(part 1 of 2)
# Autodesk Inventor assembly: BG001_trajan20_22
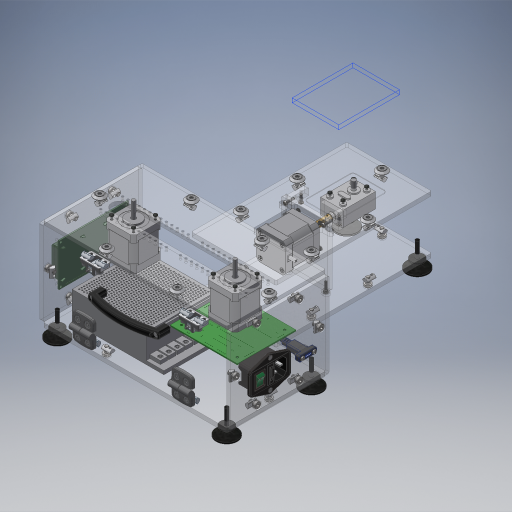
[picture p0: Inventor's stored thumbnail of the model, 512x512]
Saved by Autodesk Inventor 2023 (Build 270158000, 158)
## iProperties
Company: HTBLA Kaindorf
RuleStatus: InUse
Created: 2022-10-30
Part Number: BG001_trajan20_22
Project: Zeichenmaschine_neu
Material: Generisch
Description: Gerüst_mit_Platten
Document SubType Name: Assembly
Designer: trajan20
AfterDocNew0: iProperties-Editor_aufrufen
Author: jan
Keywords: 2022
## Documents named in this file (49)
- C:\Users\eligo\Desktop\DrawMachine\DrawMachineConstruction\inventor\BG001_trajan20_22_Zeichenmaschine_neu_Gerüst_mit_Platten.iam
- C:\Users\eligo\Desktop\DrawMachine\DrawMachineConstruction\inventor\BG000_trajan20_22_Zeichenmaschine_neu_Gestell.iam
- C:\Users\eligo\Desktop\DrawMachine\DrawMachineConstruction\inventor\BT202_trajan20_21_Zeichenmaschine_v2_getriebemotor platte unten.ipt
- C:\Users\eligo\Desktop\DrawMachine\DrawMachineConstruction\inventor\BT201_trajan20_21_Zeichenmaschine_v2_Hauptplatte unten.ipt
- C:\Users\eligo\Desktop\DrawMachine\DrawMachineConstruction\inventor\step Dateien\Steppermotor_NEMA17_17HS19-2004S1_Stepperonline.ipt
- C:\Users\eligo\Desktop\DrawMachine\DrawMachineConstruction\inventor\step Dateien\scharnier_095K2020L00.ipt
- C:\Users\eligo\Desktop\DrawMachine\DrawMachineConstruction\inventor\step Dateien\Magnetschnäpper _093094.ipt
- C:\Users\eligo\Desktop\DrawMachine\DrawMachineConstruction\inventor\step dateien\M4_Nutenstein_096214.ipt
- C:\Users\eligo\Desktop\DrawMachine\DrawMachineConstruction\inventor\BT704_trajan20_21_Zeichenmaschine_v2_Plexi_Zubau_Länge.ipt
- C:\Users\eligo\Desktop\DrawMachine\DrawMachineConstruction\inventor\BT702_trajan20_21_Zeichenmaschine_v2_Plexi_40x80.ipt
- C:\Users\eligo\Desktop\DrawMachine\DrawMachineConstruction\inventor\BT705_trajan20_21_Zeichenmaschine_v2_Plexi_Zubau_Breite.ipt
- C:\Users\eligo\Desktop\DrawMachine\DrawMachineConstruction\inventor\Normteile\de-DE\ISO 14583\ISO 14583 - M2,5x8-4.8.ipt
- C:\Users\eligo\Desktop\DrawMachine\DrawMachineConstruction\inventor\Normteile\de-DE\ISO 14583\ISO 14583 - M2,5x5-4.8.ipt
- C:\Users\eligo\Desktop\DrawMachine\DrawMachineConstruction\inventor\eigene Normteile\Senkschraube DIN 965 M4x8 51305_040_008(High).ipt
- C:\Users\eligo\Desktop\DrawMachine\DrawMachineConstruction\inventor\eigene Normteile\ART 48240 - DIN 6900-1 Z0 T M4x12_0 mm - A2_Steel.ipt
- C:\Users\eligo\Desktop\DrawMachine\DrawMachineConstruction\inventor\step dateien\M5_Nutenstein_096215.ipt
- C:\Users\eligo\Desktop\DrawMachine\DrawMachineConstruction\inventor\Normteile\de-DE\DIN 7984\DIN 7984 - M5 x 8.ipt
- C:\Users\eligo\Desktop\DrawMachine\DrawMachineConstruction\inventor\step dateien\BN 603 1229915 finishing washer M5.ipt
- C:\Users\eligo\Desktop\DrawMachine\DrawMachineConstruction\inventor\eigene Normteile\Senkschraube DIN 965 M5x14 51305_050_014(High).ipt
- C:\Users\eligo\Desktop\DrawMachine\DrawMachineConstruction\inventor\BT706_trajan20_21_Zeichenmaschine_v2_Plexi_Haupt_Display.ipt
- C:\Users\eligo\Desktop\DrawMachine\DrawMachineConstruction\inventor\step Dateien\display_lcd20x4hd44780.ipt
- C:\Users\eligo\Desktop\DrawMachine\DrawMachineConstruction\inventor\BT703_trajan20_21_Zeichenmaschine_v2_Plexi_Tür.ipt
- C:\Users\eligo\Desktop\DrawMachine\DrawMachineConstruction\inventor\BT703_B_trajan20_21_Zeichenmaschine_v2_Griff.ipt
- C:\Users\eligo\Desktop\DrawMachine\DrawMachineConstruction\inventor\Normteile\de-DE\ISO 4762(2)\ISO 4762 - M4 x 16ISO.ipt
- C:\Users\eligo\Desktop\DrawMachine\DrawMachineConstruction\inventor\Normteile\de-DE\AS 1427(03)\AS 1427 - M2 x 4(1).ipt
- C:\Users\eligo\Desktop\DrawMachine\DrawMachineConstruction\inventor\BT003_trajan20_22_Zeichenmaschine_neu_Fuß.ipt
- C:\Users\eligo\Desktop\DrawMachine\DrawMachineConstruction\inventor\BT706_trajan20_21_Zeichenmaschine_v2_Plexi_Haupt_Nothalt.ipt
- C:\Users\eligo\Desktop\DrawMachine\DrawMachineConstruction\inventor\BT801_trajan20_21_Zeichenmaschine_neu_Netzteil.ipt
- C:\Users\eligo\Desktop\DrawMachine\DrawMachineConstruction\inventor\step Dateien\Zeichenmaschine.ipt
- C:\Users\eligo\Desktop\DrawMachine\DrawMachineConstruction\inventor\step Dateien\Type-C Ext CBL - FEMALE +conn.ipt
- C:\Users\eligo\Desktop\DrawMachine\DrawMachineConstruction\inventor\step Dateien\connector-with-switch-and-fuse-3.snapshot.1\baugruppe.iam
- C:\Users\eligo\Desktop\DrawMachine\DrawMachineConstruction\inventor\Normteile\de-DE\AS 1427(03)\AS 1427 - M3 x 5(1).ipt
- C:\Users\eligo\Desktop\DrawMachine\DrawMachineConstruction\inventor\Normteile\de-DE\CNS 9671\CNS 9671 - M3 x 10.ipt
- C:\Users\eligo\Desktop\DrawMachine\DrawMachineConstruction\inventor\von gotzi\BT102_trajan20_21_Zeichenmaschine_v2_Platte Getriebemotor.ipt
- C:\Users\eligo\Desktop\DrawMachine\DrawMachineConstruction\inventor\von gotzi\BT101_trajan20_21_Zeichenmaschine_v2_Platte Stepper Motoren.ipt
- C:\Users\eligo\Desktop\DrawMachine\DrawMachineConstruction\inventor\von gotzi\BT901_goteln20_23_Zeichenmaschine_stepper_getriebe_halterung.ipt
- C:\Users\eligo\Desktop\DrawMachine\DrawMachineConstruction\inventor\Normteile\de-DE\ISO 14583\ISO 14583 - M3x12-4.8.ipt
- C:\Users\eligo\Desktop\DrawMachine\DrawMachineConstruction\inventor\BT902_goteln20_23_Zeichenmaschine_neu_stepper_getriebe_winkel.ipt
- C:\Users\eligo\Desktop\DrawMachine\DrawMachineConstruction\inventor\Normteile\de-DE\ANSI B18.3.4M(2)\ANSI B18.3.4M - M3 x 0.5 x 3(1).ipt
- C:\Users\eligo\Desktop\DrawMachine\DrawMachineConstruction\inventor\Normteile\de-DE\ANSI B18.3.4M(2)\ANSI B18.3.4M - M3 x 0.5 x 10(1).ipt
- C:\Users\eligo\Desktop\DrawMachine\DrawMachineConstruction\inventor\Normteile\de-DE\ANSI B18.3.4M(2)\ANSI B18.3.4M - M3 x 0.5 x 12(1).ipt
- C:\Users\eligo\Desktop\DrawMachine\DrawMachineConstruction\inventor\Normteile\de-DE\ISO 14583\ISO 14583 - M2,5x10-4.8.ipt
- C:\Users\eligo\Desktop\DrawMachine\DrawMachineConstruction\inventor\BT803_goteln20_22_Zeichenmaschine_neu_getriebe.ipt
- C:\Users\eligo\Desktop\DrawMachine\DrawMachineConstruction\inventor\BT804_goteln20_22_Zeichenmaschine_neu_getriebe_lagerung.ipt
- C:\Users\eligo\Desktop\DrawMachine\DrawMachineConstruction\inventor\Normteile\de-DE\DIN BEARING(1)\DIN 625 SKF - SKF 623.ipt
- C:\Users\eligo\Desktop\DrawMachine\DrawMachineConstruction\inventor\BT805_goteln20_22_Zeichenmaschine_neu_getriebe_welle_5zu2.ipt
- C:\Users\eligo\Desktop\DrawMachine\DrawMachineConstruction\inventor\BT805_goteln20_22_Zeichenmaschine_neu_getriebe_welle.ipt
- C:\Users\eligo\Desktop\DrawMachine\DrawMachineConstruction\inventor\Normteile\de-DE\BS 4168(2)\BS 4168 - M2 x 3(2).ipt
- C:\Users\eligo\Desktop\DrawMachine\DrawMachineConstruction\inventor\Normteile\de-DE\BS 4168(2)\BS 4168 - M3 x 2(2).ipt
## Components (172 placed, 48 different names)
1. BT901_goteln20_23_Zeichenmaschine_stepper_getriebe_halterung:1 — Passend:258, Passend:259, Passend:262, Passend:263, Einfügen:44, Einfügen:45, Einfügen:46, Passend:272, Passend:275, Passend:280, Passend:281, Passend:282, Passend:285, Passend:286, Passend:287, Passend:288, Passend:289, Passend:292, Passend:293
2. Schraube ISO 14583:2011(E) M3x12-4.8:1 — Passend:261, Passend:262
3. Schraube ISO 14583:2011(E) M3x12-4.8:2 — Passend:260, Passend:263, Passend:265
4. BT902_goteln20_23_Zeichenmaschine_neu_stepper_getriebe_winkel:1 — Passend:270, Passend:272, Passend:310
5. BT902_goteln20_23_Zeichenmaschine_neu_stepper_getriebe_winkel:2 — Passend:273, Passend:275, Passend:311
6. Linsenschraube mit geschmiedetem Innensechskant - Metrisch M3 x 0.5 x 12:1 — Einfügen:44
7. Linsenschraube mit geschmiedetem Innensechskant - Metrisch M3 x 0.5 x 12:2 — Einfügen:45, Passend:311
8. Linsenschraube mit geschmiedetem Innensechskant - Metrisch M3 x 0.5 x 3:3 — Einfügen:46
9. Linsenschraube mit geschmiedetem Innensechskant - Metrisch M3 x 0.5 x 10:1 — Passend:278, Passend:310
10. Linsenschraube mit geschmiedetem Innensechskant - Metrisch M3 x 0.5 x 10:2 — Passend:277
11. Steppermotor_NEMA17_17HS19-2004S1_Stepperonline:3 — Passend:280, Passend:283, Passend:284, Passend:290, Passend:291, Passend:300, Passend:304, Passend:305
12. Schraube ISO 14583:2011(E) M2,5x10-4.8:1 — Passend:281, Passend:282, Passend:283
13. Schraube ISO 14583:2011(E) M2,5x10-4.8:2 — Passend:288, Passend:291, Passend:293
14. Schraube ISO 14583:2011(E) M2,5x10-4.8:3 — Passend:284, Passend:285, Passend:286, Passend:287
15. Schraube ISO 14583:2011(E) M2,5x10-4.8:4 — Passend:289, Passend:290, Passend:292
16. BT803_goteln20_22_Zeichenmaschine_neu_getriebe:1 — Passend:294, Passend:295, Passend:296, Passend:297, Passend:298, Passend:300, Fluchtend:16, Fluchtend:17, Passend:301
17. BT804_goteln20_22_Zeichenmaschine_neu_getriebe_lagerung:1 — Fluchtend:16, Fluchtend:17, Passend:301, Einfügen:47
18. DIN 625 SKF SKF 623:1 — Einfügen:47, Passend:302, Passend:303
19. BT805_goteln20_22_Zeichenmaschine_neu_getriebe_welle_5zu2:1 — Passend:302, Passend:303, Passend:304, Passend:306, Passend:307, Passend:308, Fluchtend:18
20. BS 4168 : Teil 2 Innensechskantschrauben und Stiftschlüssel, metrische Ausführung - Spezifikation für Sechskant-Gewindestifte mit Kegelstumpf - Metrisch M3 x 2:1 — Passend:305, Passend:306
21. BS 4168 : Teil 2 Innensechskantschrauben und Stiftschlüssel, metrische Ausführung - Spezifikation für Sechskant-Gewindestifte mit Kegelstumpf - Metrisch M2 x 3:1 — Passend:307, Passend:309
22. BT805_goteln20_22_Zeichenmaschine_neu_getriebe_welle:1 — Passend:308, Fluchtend:18, Passend:309
23. BT003_trajan20_22_Zeichenmaschine_neu_Fuß:1 — Passend:205, Passend:206
24. BT003_trajan20_22_Zeichenmaschine_neu_Fuß:2 — Passend:209, Passend:211
25. BT003_trajan20_22_Zeichenmaschine_neu_Fuß:3 — Passend:207, Passend:210
26. BT003_trajan20_22_Zeichenmaschine_neu_Fuß:4 — Passend:208, Passend:212
27. BT003_trajan20_22_Zeichenmaschine_neu_Fuß:5 — Passend:214, Passend:216
28. BT003_trajan20_22_Zeichenmaschine_neu_Fuß:6 — Passend:213, Passend:215
29. BG000_trajan20_22_Zeichenmaschine_neu_Gestell:1 [sub-assembly] — Passend:2, Fluchtend:3, Fluchtend:4, Passend:3, Fluchtend:5, Fluchtend:6, Passend:14, Passend:15, Passend:16, Passend:17, Passend:18, Passend:19, Passend:20, Winkel:1, Passend:21, Passend:22, Passend:23, Passend:24, Passend:25, Passend:26, Passend:27, Passend:28, Passend:29, Passend:30, Passend:31, Passend:32, Passend:33, Passend:34, Passend:35, Passend:36, Passend:37, Passend:38, Passend:39, Passend:40, Passend:41, Passend:43, Winkel:2, Passend:45, Passend:46, Winkel:3, Winkel:4, Passend:49, Passend:50, Passend:51, Passend:52, Winkel:5, Winkel:6, Winkel:7, Winkel:8, Fluchtend:10, Fluchtend:11, Passend:74, Passend:75, Passend:76, Passend:77, Passend:85, Winkel:9, Passend:86, Passend:87, Winkel:10, Winkel:11, Passend:88, Passend:89, Winkel:12, Winkel:13, Passend:90, Winkel:14, Passend:97, Passend:98, Passend:99, Passend:100, Passend:101, Winkel:15, Winkel:16, Winkel:17, Winkel:18, Winkel:19, Passend:107, Winkel:20, Passend:108, Passend:109, Passend:110, Passend:111, Passend:112, Winkel:21, Winkel:22, Winkel:23, Winkel:24, Winkel:25, Passend:119, Winkel:26, Passend:120, Passend:121, Passend:122, Passend:123, Winkel:27, Winkel:28, Winkel:29, Winkel:30, Passend:173, Fluchtend:12, Fluchtend:13, Winkel:31, Passend:176, Passend:177, Passend:178, Passend:179, Passend:180, Passend:181, Winkel:32, Winkel:33, Winkel:34, Winkel:35, Winkel:36, Winkel:37, Passend:206, Passend:210, Passend:211, Passend:212, Passend:215, Passend:216, Passend:217, Fluchtend:14, Fluchtend:15, Passend:219, Passend:220, Passend:221, Passend:222, Passend:223, Passend:224, Passend:225, Passend:226, Winkel:38, Winkel:39, Winkel:40, Winkel:41, Winkel:42, Winkel:43, Passend:235, Passend:245
30. BT704_trajan20_21_Zeichenmaschine_v2_Plexi_Zubau_Länge:1 — Passend:27, Passend:28, Passend:29
31. BT702_trajan20_21_Zeichenmaschine_v2_Plexi_40x80:1 — Passend:33, Passend:34, Passend:35
32. BT702_trajan20_21_Zeichenmaschine_v2_Plexi_40x80:2 — Passend:36, Passend:37, Passend:38
33. BT705_trajan20_21_Zeichenmaschine_v2_Plexi_Zubau_Breite:1 — Passend:39, Passend:40, Passend:41
34. BT704_trajan20_21_Zeichenmaschine_v2_Plexi_Zubau_Länge:2 — Passend:30, Passend:31, Passend:32
35. Steppermotor_NEMA17_17HS19-2004S1_Stepperonline:2 — Passend:254, Passend:255
36. Steppermotor_NEMA17_17HS19-2004S1_Stepperonline:1 — Passend:256, Passend:257
37. Schraube ISO 14583:2011(E) M2,5x8-4.8:1 — Einfügen:36, Passend:257
38. Schraube ISO 14583:2011(E) M2,5x8-4.8:2 — Einfügen:37
39. Schraube ISO 14583:2011(E) M2,5x8-4.8:3 — Einfügen:38, Passend:256
40. Schraube ISO 14583:2011(E) M2,5x8-4.8:4 — Einfügen:39
41. Schraube ISO 14583:2011(E) M2,5x8-4.8:5 — Einfügen:40, Passend:254
42. Schraube ISO 14583:2011(E) M2,5x8-4.8:8 — Einfügen:41
43. Schraube ISO 14583:2011(E) M2,5x8-4.8:7 — Einfügen:42, Passend:255
44. Schraube ISO 14583:2011(E) M2,5x8-4.8:6 — Einfügen:43
45. Schraube ISO 14583:2011(E) M2,5x5-4.8:1 — Passend:249, Passend:253, Passend:296
46. Schraube ISO 14583:2011(E) M2,5x5-4.8:2 — Passend:252, Passend:295
47. Schraube ISO 14583:2011(E) M2,5x5-4.8:3 — Passend:251, Passend:299
48. Schraube ISO 14583:2011(E) M2,5x5-4.8:4 — Passend:250, Passend:298
49. Senkschraube DIN 965 M4x8 51305_040_008(High):1 — Passend:65, Passend:72
50. Senkschraube DIN 965 M4x8 51305_040_008(High):2 — Passend:66, Passend:71
51. Senkschraube DIN 965 M4x8 51305_040_008(High):3 — Passend:67, Passend:70
52. Senkschraube DIN 965 M4x8 51305_040_008(High):4 — Passend:68, Passend:69
53. scharnier_095K2020L00:2 — Passend:15, Passend:23, Passend:24, Passend:25, Passend:47, Passend:48, Passend:65, Passend:66, Passend:71, Passend:72, Passend:188, Passend:191, Passend:196, Passend:197
54. scharnier_095K2020L00:1 — Passend:14, Passend:21, Passend:22, Passend:26, Passend:42, Passend:44, Passend:67, Passend:68, Passend:69, Passend:70, Passend:190, Passend:198, Passend:199
55. M4_Nutenstein_096214:4 — Passend:46, Winkel:3, Passend:48
56. M4_Nutenstein_096214:3 — Passend:45, Winkel:4, Passend:47
57. M4_Nutenstein_096214:2 — Passend:43, Winkel:2, Passend:44
58. M4_Nutenstein_096214:1 — Passend:20, Winkel:1, Passend:42
59. M4_Nutenstein_096214:8 — Passend:52, Winkel:5, Passend:56, Passend:77, Passend:83
60. M4_Nutenstein_096214:5 — Passend:49, Winkel:7, Passend:53, Passend:73, Passend:74
61. M4_Nutenstein_096214:6 — Passend:50, Winkel:8, Passend:54, Passend:75, Passend:78
62. M4_Nutenstein_096214:7 — Passend:51, Winkel:6, Passend:55, Passend:76, Passend:81
63. Magnetschnäpper _093094:2 — Passend:16, Passend:18, Passend:55, Passend:56, Fluchtend:11, Passend:82, Passend:84
64. Magnetschnäpper _093094:1 — Passend:17, Passend:19, Passend:53, Passend:54, Fluchtend:10, Passend:79, Passend:80
65. ART 48240 - DIN 6900-1 Z0 T M4x12_0 mm - A2_Steel:1 — Passend:73, Passend:80
66. ART 48240 - DIN 6900-1 Z0 T M4x12_0 mm - A2_Steel:2 — Passend:78, Passend:79
67. ART 48240 - DIN 6900-1 Z0 T M4x12_0 mm - A2_Steel:3 — Passend:81, Passend:82
68. ART 48240 - DIN 6900-1 Z0 T M4x12_0 mm - A2_Steel:4 — Passend:83, Passend:84
69. BT101_trajan20_21_Zeichenmaschine_v2_Platte Stepper Motoren:2 — Einfügen:36, Einfügen:37, Einfügen:38, Einfügen:39, Einfügen:40, Einfügen:41, Einfügen:42, Einfügen:43
70. M5_Nutenstein_096215:1 — Passend:85, Winkel:9
71. M5_Nutenstein_096215:2 — Passend:86, Winkel:11
72. M5_Nutenstein_096215:3 — Passend:87, Winkel:10
73. M5_Nutenstein_096215:4 — Passend:89, Winkel:12
74. M5_Nutenstein_096215:5 — Passend:88, Winkel:13
75. M5_Nutenstein_096215:6 — Passend:90, Winkel:14
76. BN 603 1229915 finishing washer M5:1 — Passend:147
77. BN 603 1229915 finishing washer M5:2 — Passend:148
78. BN 603 1229915 finishing washer M5:3 — Passend:150
79. BN 603 1229915 finishing washer M5:4 — Passend:149
80. BN 603 1229915 finishing washer M5:5 — Passend:151
81. BN 603 1229915 finishing washer M5:6 — Passend:152
82. Senkschraube DIN 965 M5x14 51305_050_014(High):1 — Passend:148
83. Senkschraube DIN 965 M5x14 51305_050_014(High):2 — Passend:149
84. Senkschraube DIN 965 M5x14 51305_050_014(High):3 — Passend:150
85. Senkschraube DIN 965 M5x14 51305_050_014(High):4 — Passend:151
86. Senkschraube DIN 965 M5x14 51305_050_014(High):5 — Passend:152
87. Senkschraube DIN 965 M5x14 51305_050_014(High):6 — Passend:147
88. BT102_trajan20_21_Zeichenmaschine_v2_Platte Getriebemotor:2 — Passend:246, Passend:247, Passend:248, Passend:249, Passend:250, Passend:251, Passend:252, Passend:253, Passend:259, Passend:270, Passend:273, Passend:277, Passend:278, Passend:294, Passend:297, Passend:299
89. M5_Nutenstein_096215:7 — Passend:97, Winkel:17, Passend:246, Passend:247
90. M5_Nutenstein_096215:8 — Passend:98, Winkel:18
91. M5_Nutenstein_096215:9 — Passend:99, Winkel:19
92. M5_Nutenstein_096215:10 — Passend:100, Winkel:16
93. M5_Nutenstein_096215:11 — Passend:101, Winkel:15
94. BN 603 1229915 finishing washer M5:7 — Passend:169
95. BN 603 1229915 finishing washer M5:8 — Passend:172
96. BN 603 1229915 finishing washer M5:9 — Passend:171
97. BN 603 1229915 finishing washer M5:10 — Passend:170
98. BN 603 1229915 finishing washer M5:11 — Passend:168
99. Senkschraube DIN 965 M5x14 51305_050_014(High):7 — Passend:172
100. Senkschraube DIN 965 M5x14 51305_050_014(High):8 — Passend:171
101. Senkschraube DIN 965 M5x14 51305_050_014(High):9 — Passend:170, Passend:248
102. Senkschraube DIN 965 M5x14 51305_050_014(High):10 — Passend:169
103. Senkschraube DIN 965 M5x14 51305_050_014(High):11 — Passend:168
104. BT201_trajan20_21_Zeichenmaschine_v2_Hauptplatte unten:1 — Passend:3, Fluchtend:5, Fluchtend:6, Passend:113, Passend:114, Passend:115, Passend:116, Passend:117, Passend:118, Einfügen:9, Einfügen:10, Einfügen:11, Einfügen:12, Einfügen:13, Einfügen:14, Passend:205, Passend:207, Passend:208, Passend:209, Passend:218, Passend:233
105. M5_Nutenstein_096215:12 — Passend:107, Winkel:20, Passend:114
106. M5_Nutenstein_096215:13 — Passend:108, Winkel:24, Passend:118
107. M5_Nutenstein_096215:14 — Passend:109, Winkel:23, Passend:117
108. M5_Nutenstein_096215:15 — Passend:110, Winkel:25, Passend:113
109. M5_Nutenstein_096215:16 — Passend:111, Winkel:21, Passend:116
110. M5_Nutenstein_096215:17 — Passend:112, Winkel:22, Passend:115
111. DIN 7984 M5 x 8:1 — Einfügen:9
112. DIN 7984 M5 x 8:2 — Einfügen:10
113. DIN 7984 M5 x 8:3 — Einfügen:11
114. DIN 7984 M5 x 8:4 — Einfügen:12
115. DIN 7984 M5 x 8:5 — Einfügen:13
116. DIN 7984 M5 x 8:6 — Einfügen:14
117. BT202_trajan20_21_Zeichenmaschine_v2_getriebemotor platte unten:1 — Passend:2, Fluchtend:3, Fluchtend:4, Passend:124, Passend:125, Passend:126, Passend:127, Passend:128, Einfügen:15, Einfügen:16, Einfügen:17, Einfügen:18, Einfügen:19, Passend:213, Passend:214, Passend:258, Passend:260, Passend:261, Passend:264, Winkel:44
118. M5_Nutenstein_096215:18 — Passend:119, Winkel:26, Passend:124
119. M5_Nutenstein_096215:19 — Passend:120, Winkel:29, Passend:126
120. M5_Nutenstein_096215:20 — Passend:121, Winkel:30, Passend:128
121. M5_Nutenstein_096215:21 — Passend:123, Winkel:28, Passend:127
122. M5_Nutenstein_096215:22 — Passend:122, Winkel:27, Passend:125
123. DIN 7984 M5 x 8:7 — Einfügen:15
124. DIN 7984 M5 x 8:8 — Einfügen:16
125. DIN 7984 M5 x 8:9 — Einfügen:17
126. DIN 7984 M5 x 8:10 — Einfügen:18
127. DIN 7984 M5 x 8:11 — Einfügen:19
128. BT706_trajan20_21_Zeichenmaschine_v2_Plexi_Haupt_Display:1 — Passend:173, Fluchtend:12, Fluchtend:13, Passend:174, Passend:175, Passend:182, Passend:183, Passend:184, Passend:185, Passend:186, Passend:187, Einfügen:20, Einfügen:21, Einfügen:22, Einfügen:23, Einfügen:24, Einfügen:25
129. display_lcd20x4hd44780:1 — Passend:174, Passend:175, Winkel:31
130. M5_Nutenstein_096215:23 — Passend:176, Winkel:37, Passend:182
131. M5_Nutenstein_096215:24 — Passend:177, Winkel:35, Passend:187
132. M5_Nutenstein_096215:25 — Passend:178, Winkel:34, Passend:186
133. M5_Nutenstein_096215:26 — Passend:179, Winkel:36, Passend:185
134. M5_Nutenstein_096215:27 — Passend:181, Winkel:32, Passend:183
135. M5_Nutenstein_096215:28 — Passend:180, Winkel:33, Passend:184
136. DIN 7984 M5 x 8:12 — Einfügen:20
137. DIN 7984 M5 x 8:13 — Einfügen:21
138. DIN 7984 M5 x 8:14 — Einfügen:22
139. DIN 7984 M5 x 8:15 — Einfügen:23
140. DIN 7984 M5 x 8:16 — Einfügen:24
141. DIN 7984 M5 x 8:17 — Einfügen:25
142. BT703_trajan20_21_Zeichenmaschine_v2_Plexi_Tür:1 — Passend:188, Passend:190, Passend:191, Passend:192, Passend:193, Passend:194, Passend:195, Passend:200, Passend:201, Passend:202, Passend:203, Passend:204
143. BT703_B_trajan20_21_Zeichenmaschine_v2_Griff:1 — Passend:200, Passend:201, Passend:202, Einfügen:26, Einfügen:27
144. Senkschraube DIN 965 M4x8 51305_040_008(High):5 — Passend:192, Passend:198
145. Senkschraube DIN 965 M4x8 51305_040_008(High):6 — Passend:193, Passend:199
146. Senkschraube DIN 965 M4x8 51305_040_008(High):7 — Passend:194, Passend:196
147. Senkschraube DIN 965 M4x8 51305_040_008(High):8 — Passend:195, Passend:197
148. ISO 4762 M4 x 16:1 — Einfügen:26
149. ISO 4762 M4 x 16:2 — Einfügen:27
150. AS 1427 - Metrisch M2 x 4:1 — Passend:203
151. AS 1427 - Metrisch M2 x 4:2 — Passend:204
152. BT706_trajan20_21_Zeichenmaschine_v2_Plexi_Haupt_Nothalt:1 — Passend:217, Fluchtend:14, Fluchtend:15, Passend:227, Passend:228, Passend:229, Passend:230, Passend:231, Passend:232, Einfügen:28, Einfügen:29, Einfügen:30, Einfügen:31, Einfügen:32, Einfügen:33, Passend:236, Passend:237, Passend:239, Passend:240, Passend:241, Passend:244
153. M5_Nutenstein_096215:29 — Passend:221, Winkel:42, Passend:227
154. M5_Nutenstein_096215:30 — Passend:224, Winkel:40, Passend:231
155. M5_Nutenstein_096215:31 — Passend:225, Winkel:41, Passend:232
156. M5_Nutenstein_096215:32 — Passend:223, Winkel:39, Passend:229
157. M5_Nutenstein_096215:33 — Passend:222, Winkel:38, Passend:228
158. M5_Nutenstein_096215:34 — Passend:226, Winkel:43, Passend:230
159. DIN 7984 M5 x 8:23 — Einfügen:33
160. DIN 7984 M5 x 8:18 — Einfügen:28
161. DIN 7984 M5 x 8:19 — Einfügen:29
162. DIN 7984 M5 x 8:20 — Einfügen:30
163. DIN 7984 M5 x 8:21 — Einfügen:31
164. DIN 7984 M5 x 8:22 — Einfügen:32
165. Type-C Ext CBL - FEMALE +conn:1 — Passend:239, Passend:240, Passend:241, Einfügen:34, Einfügen:35
166. baugruppe:1 [sub-assembly] — Passend:236, Passend:237, Passend:242, Passend:243, Passend:244
167. AS 1427 - Metrisch M3 x 5:1 — Passend:242
168. AS 1427 - Metrisch M3 x 5:2 — Passend:243
169. CNS 9671 M3 x 10:1 — Einfügen:34
170. CNS 9671 M3 x 10:2 — Einfügen:35
171. Zeichenmaschine:1 — Passend:233, Passend:235, Passend:245
172. BT801_trajan20_21_Zeichenmaschine_neu_Netzteil:1 — Passend:218, Passend:219, Passend:220
## Relationships (382: Mate 282, Angle 44, Insert 39, Flush 17)
- [Mate]: BG000_trajan20_22_Zeichenmaschine_neu_Gestell:1 ↔ BT101_trajan20_21_Zeichenmaschine_v2_Platte Stepper Motoren:2
- [Flush]: BG000_trajan20_22_Zeichenmaschine_neu_Gestell:1 ↔ BT101_trajan20_21_Zeichenmaschine_v2_Platte Stepper Motoren:2
- [Flush]: BG000_trajan20_22_Zeichenmaschine_neu_Gestell:1 ↔ BT101_trajan20_21_Zeichenmaschine_v2_Platte Stepper Motoren:2
- Passend:2 [Mate]: BG000_trajan20_22_Zeichenmaschine_neu_Gestell:1 ↔ BT202_trajan20_21_Zeichenmaschine_v2_getriebemotor platte unten:1
- Fluchtend:3 [Flush]: BG000_trajan20_22_Zeichenmaschine_neu_Gestell:1 ↔ BT202_trajan20_21_Zeichenmaschine_v2_getriebemotor platte unten:1
- Fluchtend:4 [Flush]: BG000_trajan20_22_Zeichenmaschine_neu_Gestell:1 ↔ BT202_trajan20_21_Zeichenmaschine_v2_getriebemotor platte unten:1
- Passend:3 [Mate]: BG000_trajan20_22_Zeichenmaschine_neu_Gestell:1 ↔ BT201_trajan20_21_Zeichenmaschine_v2_Hauptplatte unten:1
- Fluchtend:5 [Flush]: BG000_trajan20_22_Zeichenmaschine_neu_Gestell:1 ↔ BT201_trajan20_21_Zeichenmaschine_v2_Hauptplatte unten:1
- Fluchtend:6 [Flush]: BG000_trajan20_22_Zeichenmaschine_neu_Gestell:1 ↔ BT201_trajan20_21_Zeichenmaschine_v2_Hauptplatte unten:1
- [Mate]: BG000_trajan20_22_Zeichenmaschine_neu_Gestell:1 ↔ BT102_trajan20_21_Zeichenmaschine_v2_Platte Getriebemotor:2
- [Flush]: BG000_trajan20_22_Zeichenmaschine_neu_Gestell:1 ↔ BT102_trajan20_21_Zeichenmaschine_v2_Platte Getriebemotor:2
- [Flush]: BG000_trajan20_22_Zeichenmaschine_neu_Gestell:1 ↔ BT102_trajan20_21_Zeichenmaschine_v2_Platte Getriebemotor:2
- [Mate]: Steppermotor_NEMA17_17HS19-2004S1_Stepperonline:2 ↔ BT101_trajan20_21_Zeichenmaschine_v2_Platte Stepper Motoren:2
- [Mate]: Steppermotor_NEMA17_17HS19-2004S1_Stepperonline:1 ↔ BT101_trajan20_21_Zeichenmaschine_v2_Platte Stepper Motoren:2
- Passend:14 [Mate]: BG000_trajan20_22_Zeichenmaschine_neu_Gestell:1 ↔ scharnier_095K2020L00:1
- Passend:15 [Mate]: BG000_trajan20_22_Zeichenmaschine_neu_Gestell:1 ↔ scharnier_095K2020L00:2
- Passend:16 [Mate]: BG000_trajan20_22_Zeichenmaschine_neu_Gestell:1 ↔ Magnetschnäpper _093094:2
- Passend:17 [Mate]: BG000_trajan20_22_Zeichenmaschine_neu_Gestell:1 ↔ Magnetschnäpper _093094:1
- Passend:18 [Mate] (26 mm): BG000_trajan20_22_Zeichenmaschine_neu_Gestell:1 ↔ Magnetschnäpper _093094:2
- Passend:19 [Mate] (26 mm): BG000_trajan20_22_Zeichenmaschine_neu_Gestell:1 ↔ Magnetschnäpper _093094:1
- Passend:20 [Mate] (0.55 mm): BG000_trajan20_22_Zeichenmaschine_neu_Gestell:1 ↔ M4_Nutenstein_096214:1
- Winkel:1 [Angle] (0 deg): BG000_trajan20_22_Zeichenmaschine_neu_Gestell:1 ↔ M4_Nutenstein_096214:1
- Passend:21 [Mate] (2.5 mm): BG000_trajan20_22_Zeichenmaschine_neu_Gestell:1 ↔ scharnier_095K2020L00:1
- Passend:22 [Mate] (2.5 mm): BG000_trajan20_22_Zeichenmaschine_neu_Gestell:1 ↔ scharnier_095K2020L00:1
- Passend:23 [Mate] (2.5 mm): BG000_trajan20_22_Zeichenmaschine_neu_Gestell:1 ↔ scharnier_095K2020L00:2
- Passend:24 [Mate] (2.5 mm): BG000_trajan20_22_Zeichenmaschine_neu_Gestell:1 ↔ scharnier_095K2020L00:2
- Passend:25 [Mate] (40 mm): BG000_trajan20_22_Zeichenmaschine_neu_Gestell:1 ↔ scharnier_095K2020L00:2
- Passend:26 [Mate] (40 mm): BG000_trajan20_22_Zeichenmaschine_neu_Gestell:1 ↔ scharnier_095K2020L00:1
- Passend:27 [Mate]: BG000_trajan20_22_Zeichenmaschine_neu_Gestell:1 ↔ BT704_trajan20_21_Zeichenmaschine_v2_Plexi_Zubau_Länge:1
- Passend:28 [Mate] (0.5 mm): BG000_trajan20_22_Zeichenmaschine_neu_Gestell:1 ↔ BT704_trajan20_21_Zeichenmaschine_v2_Plexi_Zubau_Länge:1
- Passend:29 [Mate] (0.5 mm): BG000_trajan20_22_Zeichenmaschine_neu_Gestell:1 ↔ BT704_trajan20_21_Zeichenmaschine_v2_Plexi_Zubau_Länge:1
- Passend:30 [Mate]: BG000_trajan20_22_Zeichenmaschine_neu_Gestell:1 ↔ BT704_trajan20_21_Zeichenmaschine_v2_Plexi_Zubau_Länge:2
- Passend:31 [Mate] (0.5 mm): BG000_trajan20_22_Zeichenmaschine_neu_Gestell:1 ↔ BT704_trajan20_21_Zeichenmaschine_v2_Plexi_Zubau_Länge:2
- Passend:32 [Mate] (0.5 mm): BG000_trajan20_22_Zeichenmaschine_neu_Gestell:1 ↔ BT704_trajan20_21_Zeichenmaschine_v2_Plexi_Zubau_Länge:2
- Passend:33 [Mate]: BG000_trajan20_22_Zeichenmaschine_neu_Gestell:1 ↔ BT702_trajan20_21_Zeichenmaschine_v2_Plexi_40x80:1
- Passend:34 [Mate] (0.5 mm): BG000_trajan20_22_Zeichenmaschine_neu_Gestell:1 ↔ BT702_trajan20_21_Zeichenmaschine_v2_Plexi_40x80:1
- Passend:35 [Mate] (0.5 mm): BG000_trajan20_22_Zeichenmaschine_neu_Gestell:1 ↔ BT702_trajan20_21_Zeichenmaschine_v2_Plexi_40x80:1
- Passend:36 [Mate]: BG000_trajan20_22_Zeichenmaschine_neu_Gestell:1 ↔ BT702_trajan20_21_Zeichenmaschine_v2_Plexi_40x80:2
- Passend:37 [Mate] (0.5 mm): BG000_trajan20_22_Zeichenmaschine_neu_Gestell:1 ↔ BT702_trajan20_21_Zeichenmaschine_v2_Plexi_40x80:2
- Passend:38 [Mate] (0.5 mm): BG000_trajan20_22_Zeichenmaschine_neu_Gestell:1 ↔ BT702_trajan20_21_Zeichenmaschine_v2_Plexi_40x80:2
- Passend:39 [Mate]: BG000_trajan20_22_Zeichenmaschine_neu_Gestell:1 ↔ BT705_trajan20_21_Zeichenmaschine_v2_Plexi_Zubau_Breite:1
- Passend:40 [Mate] (0.5 mm): BG000_trajan20_22_Zeichenmaschine_neu_Gestell:1 ↔ BT705_trajan20_21_Zeichenmaschine_v2_Plexi_Zubau_Breite:1
- Passend:41 [Mate] (0.5 mm): BG000_trajan20_22_Zeichenmaschine_neu_Gestell:1 ↔ BT705_trajan20_21_Zeichenmaschine_v2_Plexi_Zubau_Breite:1
- Passend:42 [Mate]: scharnier_095K2020L00:1 ↔ M4_Nutenstein_096214:1
- Passend:43 [Mate] (0.55 mm): BG000_trajan20_22_Zeichenmaschine_neu_Gestell:1 ↔ M4_Nutenstein_096214:2
- Winkel:2 [Angle] (0 deg): BG000_trajan20_22_Zeichenmaschine_neu_Gestell:1 ↔ M4_Nutenstein_096214:2
- Passend:44 [Mate]: scharnier_095K2020L00:1 ↔ M4_Nutenstein_096214:2
- Passend:45 [Mate] (0.55 mm): BG000_trajan20_22_Zeichenmaschine_neu_Gestell:1 ↔ M4_Nutenstein_096214:3
- Passend:46 [Mate] (0.55 mm): BG000_trajan20_22_Zeichenmaschine_neu_Gestell:1 ↔ M4_Nutenstein_096214:4
- Winkel:3 [Angle] (0 deg): BG000_trajan20_22_Zeichenmaschine_neu_Gestell:1 ↔ M4_Nutenstein_096214:4
- Winkel:4 [Angle] (0 deg): BG000_trajan20_22_Zeichenmaschine_neu_Gestell:1 ↔ M4_Nutenstein_096214:3
- Passend:47 [Mate]: scharnier_095K2020L00:2 ↔ M4_Nutenstein_096214:3
- Passend:48 [Mate]: scharnier_095K2020L00:2 ↔ M4_Nutenstein_096214:4
- Passend:49 [Mate] (0.55 mm): BG000_trajan20_22_Zeichenmaschine_neu_Gestell:1 ↔ M4_Nutenstein_096214:5
- Passend:50 [Mate] (0.55 mm): BG000_trajan20_22_Zeichenmaschine_neu_Gestell:1 ↔ M4_Nutenstein_096214:6
- Passend:51 [Mate] (0.55 mm): BG000_trajan20_22_Zeichenmaschine_neu_Gestell:1 ↔ M4_Nutenstein_096214:7
- Passend:52 [Mate] (0.55 mm): BG000_trajan20_22_Zeichenmaschine_neu_Gestell:1 ↔ M4_Nutenstein_096214:8
- Winkel:5 [Angle] (0 deg): BG000_trajan20_22_Zeichenmaschine_neu_Gestell:1 ↔ M4_Nutenstein_096214:8
- Winkel:6 [Angle] (0 deg): BG000_trajan20_22_Zeichenmaschine_neu_Gestell:1 ↔ M4_Nutenstein_096214:7
- Winkel:7 [Angle] (0 deg): BG000_trajan20_22_Zeichenmaschine_neu_Gestell:1 ↔ M4_Nutenstein_096214:5
- Winkel:8 [Angle] (0 deg): BG000_trajan20_22_Zeichenmaschine_neu_Gestell:1 ↔ M4_Nutenstein_096214:6
- Passend:53 [Mate] (2.15 mm): M4_Nutenstein_096214:5 ↔ Magnetschnäpper _093094:1
- Passend:54 [Mate] (2.15 mm): M4_Nutenstein_096214:6 ↔ Magnetschnäpper _093094:1
- Passend:55 [Mate] (2.15 mm): M4_Nutenstein_096214:7 ↔ Magnetschnäpper _093094:2
- Passend:56 [Mate] (2.15 mm): M4_Nutenstein_096214:8 ↔ Magnetschnäpper _093094:2
- Passend:65 [Mate]: Senkschraube DIN 965 M4x8 51305_040_008(High):1 ↔ scharnier_095K2020L00:2
- Passend:66 [Mate]: Senkschraube DIN 965 M4x8 51305_040_008(High):2 ↔ scharnier_095K2020L00:2
- Passend:67 [Mate]: Senkschraube DIN 965 M4x8 51305_040_008(High):3 ↔ scharnier_095K2020L00:1
- Passend:68 [Mate]: Senkschraube DIN 965 M4x8 51305_040_008(High):4 ↔ scharnier_095K2020L00:1
- Passend:69 [Mate]: Senkschraube DIN 965 M4x8 51305_040_008(High):4 ↔ scharnier_095K2020L00:1
- Passend:70 [Mate]: Senkschraube DIN 965 M4x8 51305_040_008(High):3 ↔ scharnier_095K2020L00:1
- Passend:71 [Mate]: Senkschraube DIN 965 M4x8 51305_040_008(High):2 ↔ scharnier_095K2020L00:2
- Passend:72 [Mate]: Senkschraube DIN 965 M4x8 51305_040_008(High):1 ↔ scharnier_095K2020L00:2
- Passend:73 [Mate]: M4_Nutenstein_096214:5 ↔ ART 48240 - DIN 6900-1 Z0 T M4x12_0 mm - A2_Steel:1
- Fluchtend:10 [Flush] (5 mm): BG000_trajan20_22_Zeichenmaschine_neu_Gestell:1 ↔ Magnetschnäpper _093094:1
- Fluchtend:11 [Flush] (5 mm): BG000_trajan20_22_Zeichenmaschine_neu_Gestell:1 ↔ Magnetschnäpper _093094:2
- Passend:74 [Mate] (2.5 mm): BG000_trajan20_22_Zeichenmaschine_neu_Gestell:1 ↔ M4_Nutenstein_096214:5
- Passend:75 [Mate] (2.5 mm): BG000_trajan20_22_Zeichenmaschine_neu_Gestell:1 ↔ M4_Nutenstein_096214:6
- Passend:76 [Mate] (2.5 mm): BG000_trajan20_22_Zeichenmaschine_neu_Gestell:1 ↔ M4_Nutenstein_096214:7
- Passend:77 [Mate] (2.5 mm): BG000_trajan20_22_Zeichenmaschine_neu_Gestell:1 ↔ M4_Nutenstein_096214:8
- Passend:78 [Mate]: M4_Nutenstein_096214:6 ↔ ART 48240 - DIN 6900-1 Z0 T M4x12_0 mm - A2_Steel:2
- Passend:79 [Mate]: Magnetschnäpper _093094:1 ↔ ART 48240 - DIN 6900-1 Z0 T M4x12_0 mm - A2_Steel:2
- Passend:80 [Mate]: Magnetschnäpper _093094:1 ↔ ART 48240 - DIN 6900-1 Z0 T M4x12_0 mm - A2_Steel:1
- Passend:81 [Mate]: M4_Nutenstein_096214:7 ↔ ART 48240 - DIN 6900-1 Z0 T M4x12_0 mm - A2_Steel:3
- Passend:82 [Mate]: Magnetschnäpper _093094:2 ↔ ART 48240 - DIN 6900-1 Z0 T M4x12_0 mm - A2_Steel:3
- Passend:83 [Mate]: M4_Nutenstein_096214:8 ↔ ART 48240 - DIN 6900-1 Z0 T M4x12_0 mm - A2_Steel:4
- Passend:84 [Mate]: Magnetschnäpper _093094:2 ↔ ART 48240 - DIN 6900-1 Z0 T M4x12_0 mm - A2_Steel:4
- Passend:85 [Mate] (0.55 mm): BG000_trajan20_22_Zeichenmaschine_neu_Gestell:1 ↔ M5_Nutenstein_096215:1
- Winkel:9 [Angle] (0 deg): BG000_trajan20_22_Zeichenmaschine_neu_Gestell:1 ↔ M5_Nutenstein_096215:1
- Passend:86 [Mate] (0.55 mm): BG000_trajan20_22_Zeichenmaschine_neu_Gestell:1 ↔ M5_Nutenstein_096215:2
- Passend:87 [Mate] (0.55 mm): BG000_trajan20_22_Zeichenmaschine_neu_Gestell:1 ↔ M5_Nutenstein_096215:3
- Winkel:10 [Angle] (0 deg): BG000_trajan20_22_Zeichenmaschine_neu_Gestell:1 ↔ M5_Nutenstein_096215:3
- Winkel:11 [Angle] (0 deg): BG000_trajan20_22_Zeichenmaschine_neu_Gestell:1 ↔ M5_Nutenstein_096215:2
- Passend:88 [Mate] (0.55 mm): BG000_trajan20_22_Zeichenmaschine_neu_Gestell:1 ↔ M5_Nutenstein_096215:5
- Passend:89 [Mate] (0.55 mm): BG000_trajan20_22_Zeichenmaschine_neu_Gestell:1 ↔ M5_Nutenstein_096215:4
- Winkel:12 [Angle] (0 deg): BG000_trajan20_22_Zeichenmaschine_neu_Gestell:1 ↔ M5_Nutenstein_096215:4
- Winkel:13 [Angle] (0 deg): BG000_trajan20_22_Zeichenmaschine_neu_Gestell:1 ↔ M5_Nutenstein_096215:5
- Passend:90 [Mate] (0.55 mm): BG000_trajan20_22_Zeichenmaschine_neu_Gestell:1 ↔ M5_Nutenstein_096215:6
- Winkel:14 [Angle] (180 deg): BG000_trajan20_22_Zeichenmaschine_neu_Gestell:1 ↔ M5_Nutenstein_096215:6
- [Mate]: BT101_trajan20_21_Zeichenmaschine_v2_Platte Stepper Motoren:2 ↔ M5_Nutenstein_096215:4
- [Mate]: BT101_trajan20_21_Zeichenmaschine_v2_Platte Stepper Motoren:2 ↔ M5_Nutenstein_096215:5
- [Mate]: BT101_trajan20_21_Zeichenmaschine_v2_Platte Stepper Motoren:2 ↔ M5_Nutenstein_096215:1
- [Mate]: BT101_trajan20_21_Zeichenmaschine_v2_Platte Stepper Motoren:2 ↔ M5_Nutenstein_096215:3
- [Mate]: BT101_trajan20_21_Zeichenmaschine_v2_Platte Stepper Motoren:2 ↔ M5_Nutenstein_096215:2
- [Mate]: BT101_trajan20_21_Zeichenmaschine_v2_Platte Stepper Motoren:2 ↔ M5_Nutenstein_096215:6
- Passend:97 [Mate] (0.55 mm): BG000_trajan20_22_Zeichenmaschine_neu_Gestell:1 ↔ M5_Nutenstein_096215:7
- Passend:98 [Mate] (0.55 mm): BG000_trajan20_22_Zeichenmaschine_neu_Gestell:1 ↔ M5_Nutenstein_096215:8
- Passend:99 [Mate] (0.55 mm): BG000_trajan20_22_Zeichenmaschine_neu_Gestell:1 ↔ M5_Nutenstein_096215:9
- Passend:100 [Mate] (0.55 mm): BG000_trajan20_22_Zeichenmaschine_neu_Gestell:1 ↔ M5_Nutenstein_096215:10
- Passend:101 [Mate] (0.55 mm): BG000_trajan20_22_Zeichenmaschine_neu_Gestell:1 ↔ M5_Nutenstein_096215:11
- Winkel:15 [Angle] (0 deg): BG000_trajan20_22_Zeichenmaschine_neu_Gestell:1 ↔ M5_Nutenstein_096215:11
- Winkel:16 [Angle] (0 deg): BG000_trajan20_22_Zeichenmaschine_neu_Gestell:1 ↔ M5_Nutenstein_096215:10
- Winkel:17 [Angle] (180 deg): BG000_trajan20_22_Zeichenmaschine_neu_Gestell:1 ↔ M5_Nutenstein_096215:7
- Winkel:18 [Angle] (0 deg): BG000_trajan20_22_Zeichenmaschine_neu_Gestell:1 ↔ M5_Nutenstein_096215:8
- Winkel:19 [Angle] (0 deg): BG000_trajan20_22_Zeichenmaschine_neu_Gestell:1 ↔ M5_Nutenstein_096215:9
- [Mate]: BT102_trajan20_21_Zeichenmaschine_v2_Platte Getriebemotor:2 ↔ M5_Nutenstein_096215:9
- [Mate]: BT102_trajan20_21_Zeichenmaschine_v2_Platte Getriebemotor:2 ↔ M5_Nutenstein_096215:8
- [Mate]: BT102_trajan20_21_Zeichenmaschine_v2_Platte Getriebemotor:2 ↔ M5_Nutenstein_096215:10
- [Mate]: BT102_trajan20_21_Zeichenmaschine_v2_Platte Getriebemotor:2 ↔ M5_Nutenstein_096215:11
- Passend:107 [Mate] (0.55 mm): BG000_trajan20_22_Zeichenmaschine_neu_Gestell:1 ↔ M5_Nutenstein_096215:12
- Winkel:20 [Angle] (0 deg): BG000_trajan20_22_Zeichenmaschine_neu_Gestell:1 ↔ M5_Nutenstein_096215:12
- Passend:108 [Mate] (0.55 mm): BG000_trajan20_22_Zeichenmaschine_neu_Gestell:1 ↔ M5_Nutenstein_096215:13
- Passend:109 [Mate] (0.55 mm): BG000_trajan20_22_Zeichenmaschine_neu_Gestell:1 ↔ M5_Nutenstein_096215:14
- Passend:110 [Mate] (0.55 mm): BG000_trajan20_22_Zeichenmaschine_neu_Gestell:1 ↔ M5_Nutenstein_096215:15
- Passend:111 [Mate] (0.55 mm): BG000_trajan20_22_Zeichenmaschine_neu_Gestell:1 ↔ M5_Nutenstein_096215:16
- Passend:112 [Mate] (0.55 mm): BG000_trajan20_22_Zeichenmaschine_neu_Gestell:1 ↔ M5_Nutenstein_096215:17
- Winkel:21 [Angle] (0 deg): BG000_trajan20_22_Zeichenmaschine_neu_Gestell:1 ↔ M5_Nutenstein_096215:16
- Winkel:22 [Angle] (0 deg): BG000_trajan20_22_Zeichenmaschine_neu_Gestell:1 ↔ M5_Nutenstein_096215:17
- Winkel:23 [Angle] (0 deg): BG000_trajan20_22_Zeichenmaschine_neu_Gestell:1 ↔ M5_Nutenstein_096215:14
- Winkel:24 [Angle] (0 deg): BG000_trajan20_22_Zeichenmaschine_neu_Gestell:1 ↔ M5_Nutenstein_096215:13
- Winkel:25 [Angle] (0 deg): BG000_trajan20_22_Zeichenmaschine_neu_Gestell:1 ↔ M5_Nutenstein_096215:15
- Passend:113 [Mate]: BT201_trajan20_21_Zeichenmaschine_v2_Hauptplatte unten:1 ↔ M5_Nutenstein_096215:15
- Passend:114 [Mate]: BT201_trajan20_21_Zeichenmaschine_v2_Hauptplatte unten:1 ↔ M5_Nutenstein_096215:12
- Passend:115 [Mate]: BT201_trajan20_21_Zeichenmaschine_v2_Hauptplatte unten:1 ↔ M5_Nutenstein_096215:17
- Passend:116 [Mate]: BT201_trajan20_21_Zeichenmaschine_v2_Hauptplatte unten:1 ↔ M5_Nutenstein_096215:16
- Passend:117 [Mate]: BT201_trajan20_21_Zeichenmaschine_v2_Hauptplatte unten:1 ↔ M5_Nutenstein_096215:14
- Passend:118 [Mate]: BT201_trajan20_21_Zeichenmaschine_v2_Hauptplatte unten:1 ↔ M5_Nutenstein_096215:13
- Passend:119 [Mate] (0.55 mm): BG000_trajan20_22_Zeichenmaschine_neu_Gestell:1 ↔ M5_Nutenstein_096215:18
- Winkel:26 [Angle] (180 deg): BG000_trajan20_22_Zeichenmaschine_neu_Gestell:1 ↔ M5_Nutenstein_096215:18
- Passend:120 [Mate] (0.55 mm): BG000_trajan20_22_Zeichenmaschine_neu_Gestell:1 ↔ M5_Nutenstein_096215:19
- Passend:121 [Mate] (0.55 mm): BG000_trajan20_22_Zeichenmaschine_neu_Gestell:1 ↔ M5_Nutenstein_096215:20
- Passend:122 [Mate] (0.55 mm): BG000_trajan20_22_Zeichenmaschine_neu_Gestell:1 ↔ M5_Nutenstein_096215:22
- Passend:123 [Mate] (0.55 mm): BG000_trajan20_22_Zeichenmaschine_neu_Gestell:1 ↔ M5_Nutenstein_096215:21
- Winkel:27 [Angle] (0 deg): BG000_trajan20_22_Zeichenmaschine_neu_Gestell:1 ↔ M5_Nutenstein_096215:22
- Winkel:28 [Angle] (0 deg): BG000_trajan20_22_Zeichenmaschine_neu_Gestell:1 ↔ M5_Nutenstein_096215:21
- Winkel:29 [Angle] (0 deg): BG000_trajan20_22_Zeichenmaschine_neu_Gestell:1 ↔ M5_Nutenstein_096215:19
- Winkel:30 [Angle] (0 deg): BG000_trajan20_22_Zeichenmaschine_neu_Gestell:1 ↔ M5_Nutenstein_096215:20
- Passend:124 [Mate]: BT202_trajan20_21_Zeichenmaschine_v2_getriebemotor platte unten:1 ↔ M5_Nutenstein_096215:18
- Passend:125 [Mate]: BT202_trajan20_21_Zeichenmaschine_v2_getriebemotor platte unten:1 ↔ M5_Nutenstein_096215:22
- Passend:126 [Mate]: BT202_trajan20_21_Zeichenmaschine_v2_getriebemotor platte unten:1 ↔ M5_Nutenstein_096215:19
- Passend:127 [Mate]: BT202_trajan20_21_Zeichenmaschine_v2_getriebemotor platte unten:1 ↔ M5_Nutenstein_096215:21
- Passend:128 [Mate]: BT202_trajan20_21_Zeichenmaschine_v2_getriebemotor platte unten:1 ↔ M5_Nutenstein_096215:20
- Einfügen:9 [Insert]: BT201_trajan20_21_Zeichenmaschine_v2_Hauptplatte unten:1 ↔ DIN 7984 M5 x 8:1
- Einfügen:10 [Insert]: BT201_trajan20_21_Zeichenmaschine_v2_Hauptplatte unten:1 ↔ DIN 7984 M5 x 8:2
- Einfügen:11 [Insert]: BT201_trajan20_21_Zeichenmaschine_v2_Hauptplatte unten:1 ↔ DIN 7984 M5 x 8:3
- Einfügen:12 [Insert]: BT201_trajan20_21_Zeichenmaschine_v2_Hauptplatte unten:1 ↔ DIN 7984 M5 x 8:4
- Einfügen:13 [Insert]: BT201_trajan20_21_Zeichenmaschine_v2_Hauptplatte unten:1 ↔ DIN 7984 M5 x 8:5
- Einfügen:14 [Insert]: BT201_trajan20_21_Zeichenmaschine_v2_Hauptplatte unten:1 ↔ DIN 7984 M5 x 8:6
- Einfügen:15 [Insert]: BT202_trajan20_21_Zeichenmaschine_v2_getriebemotor platte unten:1 ↔ DIN 7984 M5 x 8:7
- Einfügen:16 [Insert]: BT202_trajan20_21_Zeichenmaschine_v2_getriebemotor platte unten:1 ↔ DIN 7984 M5 x 8:8
- Einfügen:17 [Insert]: BT202_trajan20_21_Zeichenmaschine_v2_getriebemotor platte unten:1 ↔ DIN 7984 M5 x 8:9
- Einfügen:18 [Insert]: BT202_trajan20_21_Zeichenmaschine_v2_getriebemotor platte unten:1 ↔ DIN 7984 M5 x 8:10
- Einfügen:19 [Insert]: BT202_trajan20_21_Zeichenmaschine_v2_getriebemotor platte unten:1 ↔ DIN 7984 M5 x 8:11
- [Mate]: BT101_trajan20_21_Zeichenmaschine_v2_Platte Stepper Motoren:2 ↔ BN 603 1229915 finishing washer M5:1
- [Mate]: BT101_trajan20_21_Zeichenmaschine_v2_Platte Stepper Motoren:2 ↔ BN 603 1229915 finishing washer M5:2
- [Mate]: BT101_trajan20_21_Zeichenmaschine_v2_Platte Stepper Motoren:2 ↔ BN 603 1229915 finishing washer M5:3
- [Mate]: BT101_trajan20_21_Zeichenmaschine_v2_Platte Stepper Motoren:2 ↔ BN 603 1229915 finishing washer M5:4
- [Mate]: BT101_trajan20_21_Zeichenmaschine_v2_Platte Stepper Motoren:2 ↔ BN 603 1229915 finishing washer M5:5
- [Mate]: BT101_trajan20_21_Zeichenmaschine_v2_Platte Stepper Motoren:2 ↔ BN 603 1229915 finishing washer M5:6
- [Mate]: BT101_trajan20_21_Zeichenmaschine_v2_Platte Stepper Motoren:2 ↔ BN 603 1229915 finishing washer M5:1
- [Mate]: BT101_trajan20_21_Zeichenmaschine_v2_Platte Stepper Motoren:2 ↔ BN 603 1229915 finishing washer M5:2
- [Mate]: BT101_trajan20_21_Zeichenmaschine_v2_Platte Stepper Motoren:2 ↔ BN 603 1229915 finishing washer M5:4
- [Mate]: BT101_trajan20_21_Zeichenmaschine_v2_Platte Stepper Motoren:2 ↔ BN 603 1229915 finishing washer M5:3
- [Mate]: BT101_trajan20_21_Zeichenmaschine_v2_Platte Stepper Motoren:2 ↔ BN 603 1229915 finishing washer M5:6
- [Mate]: BT101_trajan20_21_Zeichenmaschine_v2_Platte Stepper Motoren:2 ↔ BN 603 1229915 finishing washer M5:5
- [Mate]: BT101_trajan20_21_Zeichenmaschine_v2_Platte Stepper Motoren:2 ↔ Senkschraube DIN 965 M5x14 51305_050_014(High):1
- [Mate]: BT101_trajan20_21_Zeichenmaschine_v2_Platte Stepper Motoren:2 ↔ Senkschraube DIN 965 M5x14 51305_050_014(High):2
- [Mate]: BT101_trajan20_21_Zeichenmaschine_v2_Platte Stepper Motoren:2 ↔ Senkschraube DIN 965 M5x14 51305_050_014(High):3
- [Mate]: BT101_trajan20_21_Zeichenmaschine_v2_Platte Stepper Motoren:2 ↔ Senkschraube DIN 965 M5x14 51305_050_014(High):4
- [Mate]: BT101_trajan20_21_Zeichenmaschine_v2_Platte Stepper Motoren:2 ↔ Senkschraube DIN 965 M5x14 51305_050_014(High):5
- [Mate]: BT101_trajan20_21_Zeichenmaschine_v2_Platte Stepper Motoren:2 ↔ Senkschraube DIN 965 M5x14 51305_050_014(High):6
- Passend:147 [Mate]: BN 603 1229915 finishing washer M5:1 ↔ Senkschraube DIN 965 M5x14 51305_050_014(High):6
- Passend:148 [Mate]: BN 603 1229915 finishing washer M5:2 ↔ Senkschraube DIN 965 M5x14 51305_050_014(High):1
- Passend:149 [Mate]: BN 603 1229915 finishing washer M5:4 ↔ Senkschraube DIN 965 M5x14 51305_050_014(High):2
- Passend:150 [Mate]: BN 603 1229915 finishing washer M5:3 ↔ Senkschraube DIN 965 M5x14 51305_050_014(High):3
- Passend:151 [Mate]: BN 603 1229915 finishing washer M5:5 ↔ Senkschraube DIN 965 M5x14 51305_050_014(High):4
- Passend:152 [Mate]: BN 603 1229915 finishing washer M5:6 ↔ Senkschraube DIN 965 M5x14 51305_050_014(High):5
- [Mate]: BT102_trajan20_21_Zeichenmaschine_v2_Platte Getriebemotor:2 ↔ BN 603 1229915 finishing washer M5:7
- [Mate]: BT102_trajan20_21_Zeichenmaschine_v2_Platte Getriebemotor:2 ↔ BN 603 1229915 finishing washer M5:9
- [Mate]: BT102_trajan20_21_Zeichenmaschine_v2_Platte Getriebemotor:2 ↔ BN 603 1229915 finishing washer M5:10
- [Mate]: BT102_trajan20_21_Zeichenmaschine_v2_Platte Getriebemotor:2 ↔ BN 603 1229915 finishing washer M5:8
- [Mate]: BT102_trajan20_21_Zeichenmaschine_v2_Platte Getriebemotor:2 ↔ BN 603 1229915 finishing washer M5:11
- [Mate]: BT102_trajan20_21_Zeichenmaschine_v2_Platte Getriebemotor:2 ↔ BN 603 1229915 finishing washer M5:9
- [Mate]: BT102_trajan20_21_Zeichenmaschine_v2_Platte Getriebemotor:2 ↔ BN 603 1229915 finishing washer M5:7
- [Mate]: BT102_trajan20_21_Zeichenmaschine_v2_Platte Getriebemotor:2 ↔ BN 603 1229915 finishing washer M5:8
- [Mate]: BT102_trajan20_21_Zeichenmaschine_v2_Platte Getriebemotor:2 ↔ BN 603 1229915 finishing washer M5:11
- [Mate]: BT102_trajan20_21_Zeichenmaschine_v2_Platte Getriebemotor:2 ↔ Senkschraube DIN 965 M5x14 51305_050_014(High):7
- [Mate]: BT102_trajan20_21_Zeichenmaschine_v2_Platte Getriebemotor:2 ↔ Senkschraube DIN 965 M5x14 51305_050_014(High):8
- [Mate]: BT102_trajan20_21_Zeichenmaschine_v2_Platte Getriebemotor:2 ↔ Senkschraube DIN 965 M5x14 51305_050_014(High):10
- [Mate]: BT102_trajan20_21_Zeichenmaschine_v2_Platte Getriebemotor:2 ↔ Senkschraube DIN 965 M5x14 51305_050_014(High):11
- Passend:168 [Mate]: BN 603 1229915 finishing washer M5:11 ↔ Senkschraube DIN 965 M5x14 51305_050_014(High):11
- Passend:169 [Mate]: BN 603 1229915 finishing washer M5:7 ↔ Senkschraube DIN 965 M5x14 51305_050_014(High):10
- Passend:170 [Mate]: BN 603 1229915 finishing washer M5:10 ↔ Senkschraube DIN 965 M5x14 51305_050_014(High):9
- Passend:171 [Mate]: BN 603 1229915 finishing washer M5:9 ↔ Senkschraube DIN 965 M5x14 51305_050_014(High):8
- Passend:172 [Mate]: BN 603 1229915 finishing washer M5:8 ↔ Senkschraube DIN 965 M5x14 51305_050_014(High):7
- Passend:173 [Mate]: BG000_trajan20_22_Zeichenmaschine_neu_Gestell:1 ↔ BT706_trajan20_21_Zeichenmaschine_v2_Plexi_Haupt_Display:1
- Fluchtend:12 [Flush]: BG000_trajan20_22_Zeichenmaschine_neu_Gestell:1 ↔ BT706_trajan20_21_Zeichenmaschine_v2_Plexi_Haupt_Display:1
- Fluchtend:13 [Flush]: BG000_trajan20_22_Zeichenmaschine_neu_Gestell:1 ↔ BT706_trajan20_21_Zeichenmaschine_v2_Plexi_Haupt_Display:1
- Passend:174 [Mate]: BT706_trajan20_21_Zeichenmaschine_v2_Plexi_Haupt_Display:1 ↔ display_lcd20x4hd44780:1
- Passend:175 [Mate]: BT706_trajan20_21_Zeichenmaschine_v2_Plexi_Haupt_Display:1 ↔ display_lcd20x4hd44780:1
- Winkel:31 [Angle] (0 deg): BG000_trajan20_22_Zeichenmaschine_neu_Gestell:1 ↔ display_lcd20x4hd44780:1
- Passend:176 [Mate] (0.55 mm): BG000_trajan20_22_Zeichenmaschine_neu_Gestell:1 ↔ M5_Nutenstein_096215:23
- Passend:177 [Mate] (0.55 mm): BG000_trajan20_22_Zeichenmaschine_neu_Gestell:1 ↔ M5_Nutenstein_096215:24
- Passend:178 [Mate] (0.55 mm): BG000_trajan20_22_Zeichenmaschine_neu_Gestell:1 ↔ M5_Nutenstein_096215:25
- Passend:179 [Mate] (0.55 mm): BG000_trajan20_22_Zeichenmaschine_neu_Gestell:1 ↔ M5_Nutenstein_096215:26
- Passend:180 [Mate] (0.55 mm): BG000_trajan20_22_Zeichenmaschine_neu_Gestell:1 ↔ M5_Nutenstein_096215:28
- Passend:181 [Mate] (0.55 mm): BG000_trajan20_22_Zeichenmaschine_neu_Gestell:1 ↔ M5_Nutenstein_096215:27
- Winkel:32 [Angle] (0 deg): BG000_trajan20_22_Zeichenmaschine_neu_Gestell:1 ↔ M5_Nutenstein_096215:27
- Winkel:33 [Angle] (0 deg): BG000_trajan20_22_Zeichenmaschine_neu_Gestell:1 ↔ M5_Nutenstein_096215:28
- Winkel:34 [Angle] (0 deg): BG000_trajan20_22_Zeichenmaschine_neu_Gestell:1 ↔ M5_Nutenstein_096215:25
- Winkel:35 [Angle] (0 deg): BG000_trajan20_22_Zeichenmaschine_neu_Gestell:1 ↔ M5_Nutenstein_096215:24
- Winkel:36 [Angle] (0 deg): BG000_trajan20_22_Zeichenmaschine_neu_Gestell:1 ↔ M5_Nutenstein_096215:26
- Winkel:37 [Angle] (0 deg): BG000_trajan20_22_Zeichenmaschine_neu_Gestell:1 ↔ M5_Nutenstein_096215:23
- Passend:182 [Mate]: BT706_trajan20_21_Zeichenmaschine_v2_Plexi_Haupt_Display:1 ↔ M5_Nutenstein_096215:23
- Passend:183 [Mate]: BT706_trajan20_21_Zeichenmaschine_v2_Plexi_Haupt_Display:1 ↔ M5_Nutenstein_096215:27
- Passend:184 [Mate]: BT706_trajan20_21_Zeichenmaschine_v2_Plexi_Haupt_Display:1 ↔ M5_Nutenstein_096215:28
- Passend:185 [Mate]: BT706_trajan20_21_Zeichenmaschine_v2_Plexi_Haupt_Display:1 ↔ M5_Nutenstein_096215:26
- Passend:186 [Mate]: BT706_trajan20_21_Zeichenmaschine_v2_Plexi_Haupt_Display:1 ↔ M5_Nutenstein_096215:25
- Passend:187 [Mate]: BT706_trajan20_21_Zeichenmaschine_v2_Plexi_Haupt_Display:1 ↔ M5_Nutenstein_096215:24
- Einfügen:20 [Insert]: BT706_trajan20_21_Zeichenmaschine_v2_Plexi_Haupt_Display:1 ↔ DIN 7984 M5 x 8:12
- Einfügen:21 [Insert]: BT706_trajan20_21_Zeichenmaschine_v2_Plexi_Haupt_Display:1 ↔ DIN 7984 M5 x 8:13
- Einfügen:22 [Insert]: BT706_trajan20_21_Zeichenmaschine_v2_Plexi_Haupt_Display:1 ↔ DIN 7984 M5 x 8:14
- Einfügen:23 [Insert]: BT706_trajan20_21_Zeichenmaschine_v2_Plexi_Haupt_Display:1 ↔ DIN 7984 M5 x 8:15
- Einfügen:24 [Insert]: BT706_trajan20_21_Zeichenmaschine_v2_Plexi_Haupt_Display:1 ↔ DIN 7984 M5 x 8:16
- Einfügen:25 [Insert]: BT706_trajan20_21_Zeichenmaschine_v2_Plexi_Haupt_Display:1 ↔ DIN 7984 M5 x 8:17
- Passend:188 [Mate]: scharnier_095K2020L00:2 ↔ BT703_trajan20_21_Zeichenmaschine_v2_Plexi_Tür:1
- Passend:190 [Mate]: scharnier_095K2020L00:1 ↔ BT703_trajan20_21_Zeichenmaschine_v2_Plexi_Tür:1
- Passend:191 [Mate]: scharnier_095K2020L00:2 ↔ BT703_trajan20_21_Zeichenmaschine_v2_Plexi_Tür:1
- Passend:192 [Mate]: BT703_trajan20_21_Zeichenmaschine_v2_Plexi_Tür:1 ↔ Senkschraube DIN 965 M4x8 51305_040_008(High):5
- Passend:193 [Mate]: BT703_trajan20_21_Zeichenmaschine_v2_Plexi_Tür:1 ↔ Senkschraube DIN 965 M4x8 51305_040_008(High):6
- Passend:194 [Mate]: BT703_trajan20_21_Zeichenmaschine_v2_Plexi_Tür:1 ↔ Senkschraube DIN 965 M4x8 51305_040_008(High):7
- Passend:195 [Mate]: BT703_trajan20_21_Zeichenmaschine_v2_Plexi_Tür:1 ↔ Senkschraube DIN 965 M4x8 51305_040_008(High):8
- Passend:196 [Mate]: scharnier_095K2020L00:2 ↔ Senkschraube DIN 965 M4x8 51305_040_008(High):7
- Passend:197 [Mate]: scharnier_095K2020L00:2 ↔ Senkschraube DIN 965 M4x8 51305_040_008(High):8
- Passend:198 [Mate]: scharnier_095K2020L00:1 ↔ Senkschraube DIN 965 M4x8 51305_040_008(High):5
- Passend:199 [Mate]: scharnier_095K2020L00:1 ↔ Senkschraube DIN 965 M4x8 51305_040_008(High):6
- Passend:200 [Mate]: BT703_trajan20_21_Zeichenmaschine_v2_Plexi_Tür:1 ↔ BT703_B_trajan20_21_Zeichenmaschine_v2_Griff:1
- Passend:201 [Mate]: BT703_trajan20_21_Zeichenmaschine_v2_Plexi_Tür:1 ↔ BT703_B_trajan20_21_Zeichenmaschine_v2_Griff:1
- Passend:202 [Mate]: BT703_trajan20_21_Zeichenmaschine_v2_Plexi_Tür:1 ↔ BT703_B_trajan20_21_Zeichenmaschine_v2_Griff:1
- Einfügen:26 [Insert]: BT703_B_trajan20_21_Zeichenmaschine_v2_Griff:1 ↔ ISO 4762 M4 x 16:1
- Einfügen:27 [Insert]: BT703_B_trajan20_21_Zeichenmaschine_v2_Griff:1 ↔ ISO 4762 M4 x 16:2
- Passend:203 [Mate]: BT703_trajan20_21_Zeichenmaschine_v2_Plexi_Tür:1 ↔ AS 1427 - Metrisch M2 x 4:1
- Passend:204 [Mate]: BT703_trajan20_21_Zeichenmaschine_v2_Plexi_Tür:1 ↔ AS 1427 - Metrisch M2 x 4:2